# Autodesk Inventor assembly: wheel_38mm_assembly
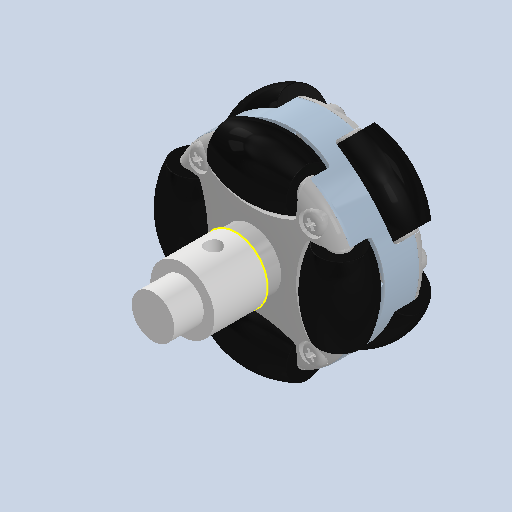
[picture p0: Inventor's stored thumbnail of the model, 512x512]
Saved by Autodesk Inventor 2025 (Build 290162000, 162)
## iProperties
Created: 2024-06-17
Part Number: wheel_38mm_assembly
Document SubType Name: Assembly
Designer: Pintu
Author: Pintu
## Documents named in this file (4)
- D:\CMC\my_inventor\ArmBo_v2\wheels\omniwheel_38mm\omniwheel_38mm\wheel_38mm_assembly.iam
- D:\CMC\my_inventor\ArmBo_v2\wheels\omniwheel_38mm\omniwheel_38mm\omniwheel_38mm.ipt
- D:\CMC\my_inventor\ArmBo_v2\wheels\omniwheel_38mm\omniwheel_38mm\hex_shaft.ipt
- D:\CMC\my_inventor\ArmBo_v2\wheels\omniwheel_38mm\omniwheel_38mm\shaft_extension.ipt
## Components (3 placed, 3 different names)
1. omniwheel_38mm:1 — Mate:1, Mate:4
2. hex_shaft:1 — Mate:1, Mate:2, Mate:3, Mate:4
3. shaft_extension:1 — Mate:2, Mate:3
## Relationships (4: Mate 4)
- Mate:1: omniwheel_38mm:1 ↔ hex_shaft:1
- Mate:2: hex_shaft:1 ↔ shaft_extension:1
- Mate:3: hex_shaft:1 ↔ shaft_extension:1
- Mate:4: omniwheel_38mm:1 ↔ hex_shaft:1
